# Autodesk Inventor assembly: Robot
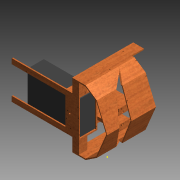
[picture p0: Inventor's stored thumbnail of the model, 180x180]
Saved by Autodesk Inventor 2014 SP1 (Build 180222100, 222)
## iProperties
Created: 2017-02-19
Part Number: Robot
Document SubType Name: Assembly
Designer: Tizon
Author: Tizon
## Documents named in this file (3)
- D:\DocsTizon\Dropbox\2016-2\Tesis 2\NNRobot\Inventor\Robot.iam
- D:\DocsTizon\Dropbox\2016-2\Tesis 2\NNRobot\Inventor\Face.ipt
- D:\DocsTizon\Dropbox\2016-2\Tesis 2\NNRobot\Inventor\Rasp.ipt
## Components (2 placed, 2 different names)
1. Face:1 — Coincidencia:1, Coincidencia:2, Nivelación:1
2. Rasp:1 — Coincidencia:1, Coincidencia:2, Nivelación:1
## Relationships (3: Mate 2, Flush 1)
- Coincidencia:1 [Mate]: Face:1 ↔ Rasp:1
- Coincidencia:2 [Mate]: Face:1 ↔ Rasp:1
- Nivelación:1 [Flush]: Face:1 ↔ Rasp:1
